# Autodesk Inventor assembly: 2DSMM-2D-Stage-MonoMotor-Layout
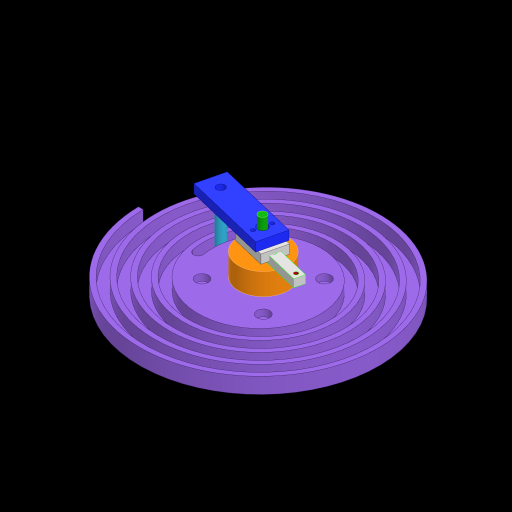
[picture p0: Inventor's stored thumbnail of the model, 512x512]
Saved by Autodesk Inventor 2024 (Build 280153000, 153)
## iProperties
Created: 2023-09-18
Part Number: 2DSMM-2D-Stage-MonoMotor-Layout
Document SubType Name: Assembly
Designer: buchmannmartin
Author: buchmannmartin
## Documents named in this file (8)
- E:\User\Dokumente\#BeneEspressoscope\2DSMM-2D-Stage-MonoMotor-Layout.iam
- E:\User\Dokumente\#BeneEspressoscope\2DSMM-Spirale.ipt
- E:\User\Dokumente\#BeneEspressoscope\2DSMM-MotorLinearadapter.ipt
- E:\User\Dokumente\#BeneEspressoscope\2DSMM-LinearachseSchiene.ipt
- E:\User\Dokumente\#BeneEspressoscope\2DSMM-LinearachseWagen.ipt
- E:\User\Dokumente\#BeneEspressoscope\2DSMM-LinearachseAdapter.ipt
- E:\User\Dokumente\#BeneEspressoscope\2DSMM-Output-DisplachementNippel.ipt
- E:\User\Dokumente\#BeneEspressoscope\2DSMM-Input-DisplachementNippel.ipt
## Components (7 placed, 7 different names)
1. 2DSMM-Spirale:1 — Passend:7, Passend:8, Übergang:1
2. 2DSMM-MotorLinearadapter:1 — Passend:4, Passend:5, Passend:6, Passend:7, Passend:8, Fluchtend:10
3. 2DSMM-LinearachseSchiene:1 — Passend:4, Passend:5, Passend:6, Fluchtend:1
4. 2DSMM-LinearachseWagen:1 — Passend:1, Passend:2, Passend:3, Fluchtend:10, Fluchtend:1, Passend:10
5. 2DSMM-LinearachseAdapter:1 — Einfügen:1, Einfügen:2, Passend:1, Passend:2, Passend:3, Passend:10
6. 2DSMM-Output-DisplachementNippel:1 — Einfügen:1, Übergang:1
7. 2DSMM-Input-DisplachementNippel:1 — Einfügen:2
## Relationships (14: Mate 9, Insert 2, Flush 2, Transitional 1)
- Einfügen:1 [Insert]: 2DSMM-LinearachseAdapter:1 ↔ 2DSMM-Output-DisplachementNippel:1
- Einfügen:2 [Insert]: 2DSMM-LinearachseAdapter:1 ↔ 2DSMM-Input-DisplachementNippel:1
- Passend:1 [Mate]: 2DSMM-LinearachseWagen:1 ↔ 2DSMM-LinearachseAdapter:1
- Passend:2 [Mate]: 2DSMM-LinearachseWagen:1 ↔ 2DSMM-LinearachseAdapter:1
- Passend:3 [Mate]: 2DSMM-LinearachseWagen:1 ↔ 2DSMM-LinearachseAdapter:1
- Passend:4 [Mate]: 2DSMM-MotorLinearadapter:1 ↔ 2DSMM-LinearachseSchiene:1
- Passend:5 [Mate]: 2DSMM-MotorLinearadapter:1 ↔ 2DSMM-LinearachseSchiene:1
- Passend:6 [Mate]: 2DSMM-MotorLinearadapter:1 ↔ 2DSMM-LinearachseSchiene:1
- Passend:7 [Mate]: 2DSMM-Spirale:1 ↔ 2DSMM-MotorLinearadapter:1
- Passend:8 [Mate] (1 mm): 2DSMM-Spirale:1 ↔ 2DSMM-MotorLinearadapter:1
- Fluchtend:10 [Flush] (-6 mm): 2DSMM-MotorLinearadapter:1 ↔ 2DSMM-LinearachseWagen:1
- Fluchtend:1 [Flush]: 2DSMM-LinearachseSchiene:1 ↔ 2DSMM-LinearachseWagen:1
- Passend:10 [Mate]: 2DSMM-LinearachseWagen:1 ↔ 2DSMM-LinearachseAdapter:1
- Übergang:1 [Transitional]: 2DSMM-Spirale:1 ↔ 2DSMM-Output-DisplachementNippel:1
